# Autodesk Inventor assembly: FullBoard
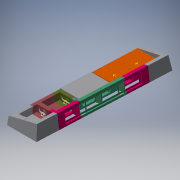
[picture p0: Inventor's stored thumbnail of the model, 180x180]
Saved by Autodesk Inventor 2019 (Build 230136000, 136)
## iProperties
Created: 2019-01-04
Part Number: FullBoard
Document SubType Name: Assembly
Designer: james
Author: james
## Documents named in this file (15)
- F:\JimsDesign\4089DriversStation\FullBoard.iam
- F:\JimsDesign\4089DriversStation\ControlPlate.ipt
- F:\JimsDesign\4089DriversStation\CPLRightOne.ipt
- F:\JimsDesign\4089DriversStation\CPLRightTwo.ipt
- F:\JimsDesign\4089DriversStation\CPLRightThree.ipt
- F:\JimsDesign\4089DriversStation\CPLLeftThree.ipt
- F:\JimsDesign\4089DriversStation\CPLLeftTwo.ipt
- F:\JimsDesign\4089DriversStation\CPLLeftOne.ipt
- F:\JimsDesign\4089DriversStation\SurfaceBook2.ipt
- F:\JimsDesign\4089DriversStation\CPURightOneNew.ipt
- F:\JimsDesign\4089DriversStation\CPULeftOne.ipt
- F:\JimsDesign\4089DriversStation\CPURightTwo.ipt
- F:\JimsDesign\4089DriversStation\CPULeftTwo.ipt
- F:\JimsDesign\4089DriversStation\CPURightThree.ipt
- F:\JimsDesign\4089DriversStation\CPULeftThree.ipt
## Components (16 placed, 14 different names)
1. ControlPlate:1 — Mate:5, Mate:8, Flush:4, Mate:13
2. CPLRightOne:1 — Mate:5, Mate:6, Flush:2, Flush:3, Mate:15, Flush:13, Flush:14, Mate:17, Mate:18
3. CPLRightTwo:1 — Mate:6, Flush:2, Flush:3, Mate:7, Mate:9, Flush:5, Flush:6, Mate:23, Flush:17
4. ControlPlate:2 — Mate:7, Mate:8, Flush:4, Mate:20
5. CPLRightThree:1 — Mate:9, Flush:5, Flush:6, Mate:10, Flush:7, Flush:8
6. CPLLeftThree:1 — Mate:10, Flush:7, Flush:8, Mate:11, Flush:9, Flush:10, Mate:14, Mate:19, Mate:21, Flush:19
7. CPLLeftTwo:1 — Mate:11, Flush:9, Flush:10, Mate:12, Flush:11, Flush:12, Mate:20
8. CPLLeftOne:1 — Mate:12, Flush:11, Flush:12, Mate:13, Mate:22, Flush:15, Flush:16
9. SurfaceBook2:1 — Mate:14, Mate:19, Mate:21
10. CPURightOneNew:1 — Mate:15, Flush:13, Flush:14, Mate:16, Mate:24
11. ControlPlate:3 — Mate:16, Mate:17, Mate:18
12. CPULeftOne:1 — Mate:22, Flush:15, Flush:16, Mate:25
13. CPURightTwo:1 — Mate:23, Flush:17, Mate:24, Flush:18, Flush:20, Mate:26, Flush:21
14. CPULeftTwo:1 — Flush:18, Flush:19, Mate:25, Flush:23
15. CPURightThree:1 — Flush:20, Mate:26, Flush:21, Mate:27, Flush:22
16. CPULeftThree:1 — Mate:27, Flush:22, Flush:23
## Relationships (45: Mate 23, Flush 22)
- Mate:5: ControlPlate:1 ↔ CPLRightOne:1
- Mate:6: CPLRightOne:1 ↔ CPLRightTwo:1
- Flush:2: CPLRightOne:1 ↔ CPLRightTwo:1
- Flush:3: CPLRightOne:1 ↔ CPLRightTwo:1
- Mate:7: CPLRightTwo:1 ↔ ControlPlate:2
- Mate:8: ControlPlate:1 ↔ ControlPlate:2
- Flush:4: ControlPlate:1 ↔ ControlPlate:2
- Mate:9: CPLRightTwo:1 ↔ CPLRightThree:1
- Flush:5: CPLRightTwo:1 ↔ CPLRightThree:1
- Flush:6: CPLRightTwo:1 ↔ CPLRightThree:1
- Mate:10: CPLRightThree:1 ↔ CPLLeftThree:1
- Flush:7: CPLRightThree:1 ↔ CPLLeftThree:1
- Flush:8: CPLRightThree:1 ↔ CPLLeftThree:1
- Mate:11: CPLLeftThree:1 ↔ CPLLeftTwo:1
- Flush:9: CPLLeftThree:1 ↔ CPLLeftTwo:1
- Flush:10: CPLLeftThree:1 ↔ CPLLeftTwo:1
- Mate:12: CPLLeftTwo:1 ↔ CPLLeftOne:1
- Flush:11: CPLLeftTwo:1 ↔ CPLLeftOne:1
- Flush:12: CPLLeftTwo:1 ↔ CPLLeftOne:1
- Mate:13: ControlPlate:1 ↔ CPLLeftOne:1
- Mate:14: CPLLeftThree:1 ↔ SurfaceBook2:1
- Mate:15: CPLRightOne:1 ↔ CPURightOneNew:1
- Flush:13: CPLRightOne:1 ↔ CPURightOneNew:1
- Flush:14: CPLRightOne:1 ↔ CPURightOneNew:1
- Mate:16: CPURightOneNew:1 ↔ ControlPlate:3
- Mate:17: CPLRightOne:1 ↔ ControlPlate:3
- Mate:18: CPLRightOne:1 ↔ ControlPlate:3
- Mate:19: CPLLeftThree:1 ↔ SurfaceBook2:1
- Mate:20: ControlPlate:2 ↔ CPLLeftTwo:1
- Mate:21: CPLLeftThree:1 ↔ SurfaceBook2:1
- Mate:22: CPLLeftOne:1 ↔ CPULeftOne:1
- Flush:15: CPLLeftOne:1 ↔ CPULeftOne:1
- Flush:16: CPLLeftOne:1 ↔ CPULeftOne:1
- Mate:23: CPLRightTwo:1 ↔ CPURightTwo:1
- Flush:17: CPLRightTwo:1 ↔ CPURightTwo:1
- Mate:24: CPURightOneNew:1 ↔ CPURightTwo:1
- Flush:18: CPURightTwo:1 ↔ CPULeftTwo:1
- Flush:19: CPLLeftThree:1 ↔ CPULeftTwo:1
- Mate:25: CPULeftOne:1 ↔ CPULeftTwo:1
- Flush:20: CPURightTwo:1 ↔ CPURightThree:1
- Mate:26: CPURightTwo:1 ↔ CPURightThree:1
- Flush:21: CPURightTwo:1 ↔ CPURightThree:1
- Mate:27: CPURightThree:1 ↔ CPULeftThree:1
- Flush:22: CPURightThree:1 ↔ CPULeftThree:1
- Flush:23: CPULeftTwo:1 ↔ CPULeftThree:1
